# Autodesk Inventor assembly: ProbeHead V5 - Assembly
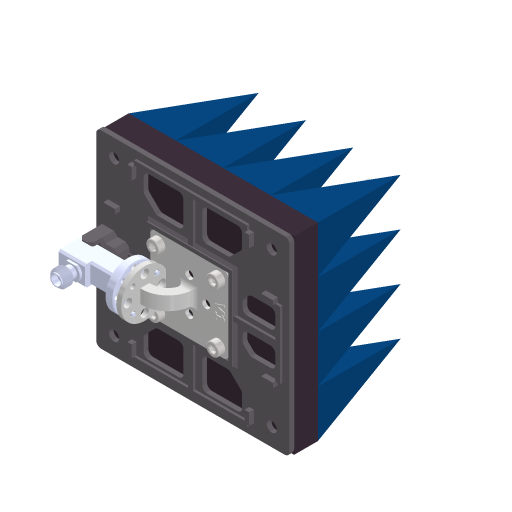
[picture p0: Inventor's stored thumbnail of the model, 512x512]
Saved by Autodesk Inventor 2023.2 (Build 272271000, 271)
## iProperties
Created: 2024-02-09
Part Number: ProbeHead V5 - Assembly
Document SubType Name: Assembly
Designer: Nils Bade
Author: Nils Bade
## Documents named in this file (9)
- C:\Users\nilsb\Documents\Inventor\Projektarbeit-Bade\RatRig_modified\ProbeHead\ProbeAntennas\OERWG_Probe_Plate.iam
- C:\Users\nilsb\Documents\Inventor\Projektarbeit-Bade\RatRig_Standards\Hex Nut - M3 v2.ipt
- C:\Users\nilsb\Documents\Inventor\Projektarbeit-Bade\Enclosure\Absorber\Absorber - IHF-Mini.ipt
- C:\Users\nilsb\Documents\Inventor\Projektarbeit-Bade\RatRig_modified\ProbeHead\ProbeAntennas\ProbeAntenna_AdapterPlate_V1.ipt
- C:\Users\nilsb\Documents\Inventor\Projektarbeit-Bade\RatRig_modified\ProbeHead\ProbeAntennas\ProbeAntenna_AdapterRWG_V1_Assembled.iam
- C:\Users\nilsb\Documents\Inventor\Projektarbeit-Bade\RatRig_Standards\Cap Head Screw M3x8 v2.ipt
- C:\Users\nilsb\Documents\Inventor\Projektarbeit-Bade\RatRig_modified\ProbeHead\ProbeAntennas\IHFStandardParts\RWG-V_Band Backingplate.ipt
- C:\Users\nilsb\Documents\Inventor\Projektarbeit-Bade\RatRig_modified\ProbeHead\ProbeAntennas\ProbeAntenna_V3_Assembled.ipt
- C:\Users\nilsb\Documents\Inventor\Projektarbeit-Bade\RatRig_modified\ProbeHead\Wire2Probe_Eravant_SWC-15VF-R1-V.ipt
## Components (29 placed, 8 different names)
1. ProbeAntenna_AdapterPlate_V1:1 — Passend:107, Passend:108, Passend:109, Passend:121, Passend:122, Passend:123, Passend:124
2. ProbeAntenna_AdapterRWG_V1_Assembled:1 [sub-assembly] — Passend:107, Passend:108, Passend:109, Passend:113, Passend:114, Passend:115, Passend:116, Passend:117, Passend:118, Passend:119, Passend:120, Passend:133, Passend:134, Passend:135, Passend:139, Winkel:1, Passend:140
3. Cap Head Screw M3x8 v2:1 — Passend:113, Passend:119, Passend:128
4. Cap Head Screw M3x8 v2:2 — Passend:114, Passend:118, Passend:127
5. Cap Head Screw M3x8 v2:3 — Passend:116, Passend:120, Passend:125
6. Cap Head Screw M3x8 v2:4 — Passend:115, Passend:117, Passend:126
7. Hex Nut - M3 v2:5 — Passend:122, Passend:127
8. Hex Nut - M3 v2:6 — Passend:121, Passend:126
9. Hex Nut - M3 v2:7 — Passend:123, Passend:128
10. Hex Nut - M3 v2:8 — Passend:124, Passend:125
11. RWG-V_Band Backingplate:1 — Passend:133, Passend:134, Passend:135
12. ProbeAntenna_V3_Assembled:1
13. Wire2Probe_Eravant_SWC-15VF-R1-V:1 — Passend:139, Winkel:1, Passend:140
14. Absorber - IHF-Mini:1
15. Absorber - IHF-Mini:18
16. Absorber - IHF-Mini:19
17. Absorber - IHF-Mini:4
18. Absorber - IHF-Mini:22
19. Absorber - IHF-Mini:21
20. Absorber - IHF-Mini:7
21. Absorber - IHF-Mini:8
22. Absorber - IHF-Mini:23
23. Absorber - IHF-Mini:24
24. Absorber - IHF-Mini:11
25. Absorber - IHF-Mini:17
26. Absorber - IHF-Mini:25
27. Absorber - IHF-Mini:26
28. Absorber - IHF-Mini:27
29. Absorber - IHF-Mini:16
## Component patterns: (16 elements, first: Absorber - IHF-Mini:1)
## Relationships (28: Mate 27, Angle 1)
- Passend:107 [Mate]: ProbeAntenna_AdapterPlate_V1:1 ↔ ProbeAntenna_AdapterRWG_V1_Assembled:1
- Passend:108 [Mate]: ProbeAntenna_AdapterPlate_V1:1 ↔ ProbeAntenna_AdapterRWG_V1_Assembled:1
- Passend:109 [Mate]: ProbeAntenna_AdapterPlate_V1:1 ↔ ProbeAntenna_AdapterRWG_V1_Assembled:1
- Passend:113 [Mate]: ProbeAntenna_AdapterRWG_V1_Assembled:1 ↔ Cap Head Screw M3x8 v2:1
- Passend:114 [Mate]: ProbeAntenna_AdapterRWG_V1_Assembled:1 ↔ Cap Head Screw M3x8 v2:2
- Passend:115 [Mate]: ProbeAntenna_AdapterRWG_V1_Assembled:1 ↔ Cap Head Screw M3x8 v2:4
- Passend:116 [Mate]: ProbeAntenna_AdapterRWG_V1_Assembled:1 ↔ Cap Head Screw M3x8 v2:3
- Passend:117 [Mate]: ProbeAntenna_AdapterRWG_V1_Assembled:1 ↔ Cap Head Screw M3x8 v2:4
- Passend:118 [Mate]: ProbeAntenna_AdapterRWG_V1_Assembled:1 ↔ Cap Head Screw M3x8 v2:2
- Passend:119 [Mate]: ProbeAntenna_AdapterRWG_V1_Assembled:1 ↔ Cap Head Screw M3x8 v2:1
- Passend:120 [Mate]: ProbeAntenna_AdapterRWG_V1_Assembled:1 ↔ Cap Head Screw M3x8 v2:3
- Passend:121 [Mate]: ProbeAntenna_AdapterPlate_V1:1 ↔ Hex Nut - M3 v2:6
- Passend:122 [Mate]: ProbeAntenna_AdapterPlate_V1:1 ↔ Hex Nut - M3 v2:5
- Passend:123 [Mate]: ProbeAntenna_AdapterPlate_V1:1 ↔ Hex Nut - M3 v2:7
- Passend:124 [Mate]: ProbeAntenna_AdapterPlate_V1:1 ↔ Hex Nut - M3 v2:8
- Passend:125 [Mate]: Cap Head Screw M3x8 v2:3 ↔ Hex Nut - M3 v2:8
- Passend:126 [Mate]: Cap Head Screw M3x8 v2:4 ↔ Hex Nut - M3 v2:6
- Passend:127 [Mate]: Cap Head Screw M3x8 v2:2 ↔ Hex Nut - M3 v2:5
- Passend:128 [Mate]: Cap Head Screw M3x8 v2:1 ↔ Hex Nut - M3 v2:7
- Passend:133 [Mate]: ProbeAntenna_AdapterRWG_V1_Assembled:1 ↔ RWG-V_Band Backingplate:1
- Passend:134 [Mate]: ProbeAntenna_AdapterRWG_V1_Assembled:1 ↔ RWG-V_Band Backingplate:1
- Passend:135 [Mate]: ProbeAntenna_AdapterRWG_V1_Assembled:1 ↔ RWG-V_Band Backingplate:1
- [Mate]: ProbeAntenna_AdapterRWG_V1_Assembled:1 ↔ ProbeAntenna_V3_Assembled:1
- [Mate]: ProbeAntenna_AdapterRWG_V1_Assembled:1 ↔ ProbeAntenna_V3_Assembled:1
- [Mate]: ProbeAntenna_AdapterRWG_V1_Assembled:1 ↔ ProbeAntenna_V3_Assembled:1
- Passend:139 [Mate]: ProbeAntenna_AdapterRWG_V1_Assembled:1 ↔ Wire2Probe_Eravant_SWC-15VF-R1-V:1
- Winkel:1 [Angle] (0 deg): ProbeAntenna_AdapterRWG_V1_Assembled:1 ↔ Wire2Probe_Eravant_SWC-15VF-R1-V:1
- Passend:140 [Mate]: ProbeAntenna_AdapterRWG_V1_Assembled:1 ↔ Wire2Probe_Eravant_SWC-15VF-R1-V:1
